# Autodesk Inventor assembly: 02CybertruckAssembly
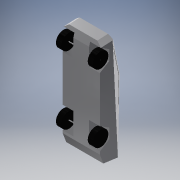
[picture p0: Inventor's stored thumbnail of the model, 180x180]
Saved by Autodesk Inventor 2018 (Build 220112000, 112)
## iProperties
Created: 2020-06-23
Part Number: 02CybertruckAssembly
Document SubType Name: Assembly
Designer: Ivan
Author: Ivan
## Documents named in this file (3)
- C:\Users\Ivan\Documents\GitHub\Proyectos980\Modelos3D\02CybertruckAssembly.iam
- C:\Users\Ivan\Documents\GitHub\Proyectos980\Modelos3D\02Cybertruck.ipt
- C:\Users\Ivan\Documents\GitHub\Proyectos980\Modelos3D\02CybertruckWheels.ipt
## Components (5 placed, 2 different names)
1. 02Cybertruck:1 — Mate:1, Mate:2, Insert:1, Insert:2, Insert:3
2. 02CybertruckWheels:1 — Mate:1, Mate:2
3. 02CybertruckWheels:2 — Insert:1
4. 02CybertruckWheels:3 — Insert:3
5. 02CybertruckWheels:4 — Insert:2
## Relationships (5: Insert 3, Mate 2)
- Mate:1: 02Cybertruck:1 ↔ 02CybertruckWheels:1
- Mate:2: 02Cybertruck:1 ↔ 02CybertruckWheels:1
- Insert:1: 02Cybertruck:1 ↔ 02CybertruckWheels:2
- Insert:2: 02Cybertruck:1 ↔ 02CybertruckWheels:4
- Insert:3: 02Cybertruck:1 ↔ 02CybertruckWheels:3
